# Autodesk Inventor assembly: Casing_assembly
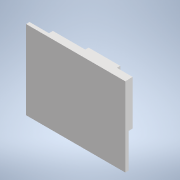
[picture p0: Inventor's stored thumbnail of the model, 180x180]
Saved by Autodesk Inventor 2020 (Build 240168000, 168)
## iProperties
Created: 2019-07-15
Part Number: Casing_assembly
Document SubType Name: Assembly
Designer: Senior Design
Author: Senior Design
## Documents named in this file (3)
- C:\Users\Senior Design\Documents\Casing_assembly.iam
- C:\Users\Senior Design\Documents\LCDScreen.ipt
- C:\Users\Senior Design\Documents\nuc_w_bracket.iam
## Components (2 placed, 2 different names)
1. LCDScreen:1 — Flush:1, Mate:12, Mate:13, Mate:14, Mate:15, Mate:16
2. nuc_w_bracket:1 [sub-assembly] — Mate:14, Mate:15, Mate:16
## Relationships (6: Mate 5, Flush 1)
- Flush:1: LCDScreen:1
- Mate:12: LCDScreen:1
- Mate:13: LCDScreen:1
- Mate:14: LCDScreen:1 ↔ nuc_w_bracket:1
- Mate:15: LCDScreen:1 ↔ nuc_w_bracket:1
- Mate:16: LCDScreen:1 ↔ nuc_w_bracket:1
